# Autodesk Inventor assembly: Assembly1
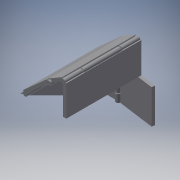
[picture p0: Inventor's stored thumbnail of the model, 180x180]
Saved by Autodesk Inventor 2019 (Build 230136000, 136)
## iProperties
Created: 2018-08-03
Part Number: Assembly1
Document SubType Name: Assembly
Designer: Ge Shi
Author: Ge Shi
## Documents named in this file (8)
- D:\hive\projects\foldingBaby\v2\Assembly1.iam
- D:\hive\projects\foldingBaby\v2\backPlate_splitDiagonal.ipt
- D:\hive\projects\foldingBaby\v2\innerFrontPlate.ipt
- D:\hive\projects\foldingBaby\v2\innerLeftRightPlate.ipt
- D:\hive\projects\foldingBaby\v2\leftRightPlate.ipt
- D:\hive\projects\foldingBaby\v2\outerFrontPlate.ipt
- D:\hive\projects\foldingBaby\v2\topBottomPlate.ipt
- D:\hive\projects\foldingBaby\v2\prototype2dims.ipt
## Components (6 placed, 6 different names)
1. backPlate_splitDiagonal:1 — Mate:1, Mate:2, Mate:5, Mate:6, Mate:14, Angle:1
2. innerFrontPlate:1 — Mate:7, Mate:8, Mate:11, Mate:12
3. innerLeftRightPlate:1 — Mate:11, Mate:12, Mate:14
4. outerFrontPlate:1 — Mate:3, Mate:4
5. topBottomPlate:1 — Mate:1, Mate:2, Mate:3, Mate:4, Angle:1
6. leftRightPlate:2 — Mate:5, Mate:6, Mate:7, Mate:8
## Relationships (12: Mate 11, Angle 1)
- Mate:1: backPlate_splitDiagonal:1 ↔ topBottomPlate:1
- Mate:2 (0.75 mm): backPlate_splitDiagonal:1 ↔ topBottomPlate:1
- Mate:3: outerFrontPlate:1 ↔ topBottomPlate:1
- Mate:4 (0.75 mm): outerFrontPlate:1 ↔ topBottomPlate:1
- Mate:5: backPlate_splitDiagonal:1 ↔ leftRightPlate:2
- Mate:6 (0.75 mm): backPlate_splitDiagonal:1 ↔ leftRightPlate:2
- Mate:7: innerFrontPlate:1 ↔ leftRightPlate:2
- Mate:8: innerFrontPlate:1 ↔ leftRightPlate:2
- Mate:11: innerFrontPlate:1 ↔ innerLeftRightPlate:1
- Mate:12 (0.75 mm): innerFrontPlate:1 ↔ innerLeftRightPlate:1
- Mate:14: backPlate_splitDiagonal:1 ↔ innerLeftRightPlate:1
- Angle:1 (-90 deg): backPlate_splitDiagonal:1 ↔ topBottomPlate:1
## Named parameters: clearance = 1.5 mm
